# Autodesk Inventor assembly: Estructura_bk02
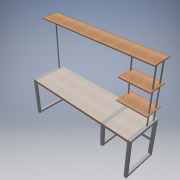
[picture p0: Inventor's stored thumbnail of the model, 180x180]
Saved by Autodesk Inventor 2016 (Build 200138000, 138)
## iProperties
Created: 2018-06-24
Part Number: Estructura_bk02
Document SubType Name: Assembly
Designer: damia
_SolveAssemblyDoc: Frame Generator Solve Assembly
_Version: 15.0.0
Author: damia
## Documents named in this file (10)
- C:\Users\damia\Documents\Inventor\escritorio_Damian\Estructura_bk02.iam
- C:\Users\damia\Documents\Inventor\Escritorio_Damian\Esqueleto.ipt
- C:\Users\damia\Documents\Inventor\Escritorio_Damian\Estructura\Frame\Frame0002.iam
- C:\Users\damia\Documents\Inventor\Escritorio_Damian\Part42.ipt
- C:\Users\damia\Documents\Inventor\Escritorio_Damian\VidrioChico.ipt
- C:\Users\damia\Documents\Inventor\Escritorio_Damian\tablero_chico.ipt
- C:\Users\damia\Documents\Inventor\Escritorio_Damian\tablero_granded.ipt
- C:\Users\damia\Documents\Inventor\Escritorio_Damian\Esqueleto_Estantes.ipt
- C:\Users\damia\Documents\Inventor\Escritorio_Damian\Estante01.ipt
- C:\Users\damia\Documents\Inventor\Escritorio_Damian\estante02.ipt
## Components (10 placed, 9 different names)
1. Esqueleto:1 — Mate:1, Mate:2
2. Frame0002:1 [sub-assembly] — Flush:7, Flush:8, Flush:9, Mate:7, Flush:12
3. tablero_granded:1
4. tablero_chico:1
5. VidrioGrande:1
6. VidrioChico:1
7. Esqueleto_Estantes:1 — Flush:7, Flush:8
8. Estante01:1 — Flush:9, Flush:10, Flush:11
9. Estante01:2 — Flush:10, Flush:11, Mate:7
10. estante02:1 — Flush:12
## Relationships (19: Flush 12, Mate 7)
- Mate:1: Esqueleto:1
- Mate:2: Esqueleto:1
- [Flush]: tablero_granded:1 ↔ VidrioGrande:1
- [Flush]: tablero_granded:1 ↔ VidrioGrande:1
- [Flush]: tablero_chico:1 ↔ VidrioChico:1
- [Flush]: tablero_chico:1 ↔ VidrioChico:1
- [Flush]: Frame0002:1 ↔ tablero_chico:1
- [Mate]: Frame0002:1 ↔ tablero_chico:1
- [Mate]: Frame0002:1 ↔ tablero_chico:1
- [Mate]: Frame0002:1 ↔ tablero_granded:1
- [Flush]: Frame0002:1 ↔ tablero_granded:1
- [Mate]: Frame0002:1 ↔ tablero_granded:1
- Flush:7: Frame0002:1 ↔ Esqueleto_Estantes:1
- Flush:8: Frame0002:1 ↔ Esqueleto_Estantes:1
- Flush:9: Frame0002:1 ↔ Estante01:1
- Flush:10: Estante01:1 ↔ Estante01:2
- Flush:11: Estante01:1 ↔ Estante01:2
- Mate:7: Frame0002:1 ↔ Estante01:2
- Flush:12: Frame0002:1 ↔ estante02:1
## Named parameters: d14_d8 = 0 mm, d16_d6 = 0 mm, d17_d7 = 0 mm
